# Autodesk Inventor assembly: 胴体_1
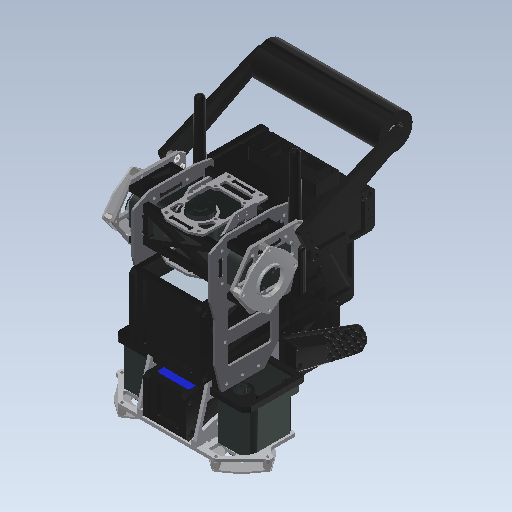
[picture p0: Inventor's stored thumbnail of the model, 512x512]
Saved by Autodesk Inventor 2020.4 (Build 244396000, 396)
## iProperties
Created: 2016-05-03
Part Number: 胴体_1
Document SubType Name: Assembly
Designer: hiroaki
Mass: 1394.39 g
Surface Area: 4542.63 cm^2
Volume: 847.153 cm^3
Density: 1.64598 g/cm^3
Author: hiroaki
## Documents named in this file (25)
- C:\Users\Masato\Documents\Inventor\CIT Brains_Inventor\OpenPlatform_ver3_0\上半身\胴体\胴体_1.iam
- C:\Users\Masato\Documents\Inventor\CIT Brains_Inventor\OpenPlatform_ver3_0\Ready_Made\B3M11xx.ipt
- C:\Users\Masato\Documents\Inventor\CIT Brains_Inventor\OpenPlatform_ver3_0\Ready_Made\B3M10xx.ipt
- C:\Users\Masato\Documents\Inventor\CIT Brains_Inventor\OpenPlatform_ver3_0\上半身\胴体\胴体_メインフレーム_1_1.ipt
- C:\Users\Masato\Documents\Inventor\CIT Brains_Inventor\OpenPlatform_ver3_0\下半身\付け根ロール\付け根ロール_サブフレーム_1_3.ipt
- C:\Users\Masato\Documents\Inventor\CIT Brains_Inventor\OpenPlatform_ver3_0\上半身\胴体\胴体_メインフレーム_1_2.ipt
- C:\Users\Masato\Documents\Inventor\CIT Brains_Inventor\OpenPlatform_ver3_0\上半身\胴体\胴体_サブフレーム_1_1.ipt
- C:\Users\Masato\Documents\Inventor\CIT Brains_Inventor\OpenPlatform_ver3_0\上半身\胴体\胴体_サブフレーム_1_2.ipt
- C:\Users\Masato\Documents\Inventor\CIT Brains_Inventor\OpenPlatform_ver3_0\上半身\胴体\胴体_サブフレーム_1_3.ipt
- C:\Users\Masato\Documents\Inventor\CIT Brains_Inventor\OpenPlatform_ver3_0\上半身\胴体\胴体_サブフレーム_1_4.ipt
- C:\Users\Masato\Documents\Inventor\CIT Brains_Inventor\OpenPlatform_ver3_0\上半身\胴体\胴体_サブフレーム_1_1_MIR.ipt
- C:\Users\Masato\Documents\Inventor\CIT Brains_Inventor\OpenPlatform_ver3_0\上半身\胴体\胴体_メインフレーム_1_12.ipt
- C:\Users\Masato\Documents\Inventor\CIT Brains_Inventor\OpenPlatform_ver3_0\上半身\胴体\胴体_メインフレーム_1_13.ipt
- C:\Users\Masato\Documents\Inventor\CIT Brains_Inventor\OpenPlatform_ver3_0\Ready_Made\MSU-306-03.ipt
- C:\Users\Masato\Documents\Inventor\CIT Brains_Inventor\OpenPlatform_ver3_0\上半身\胴体\胴体_サブフレーム_1_12.ipt
- C:\Users\Masato\Documents\Inventor\CIT Brains_Inventor\OpenPlatform_ver3_0\上半身\胴体\胴体_サブフレーム_1_4_MIR.ipt
- C:\Users\Masato\Documents\Inventor\CIT Brains_Inventor\OpenPlatform_ver3_0\上半身\胴体\RearBumper_Lower.ipt
- C:\Users\Masato\Documents\Inventor\CIT Brains_Inventor\OpenPlatform_ver3_0\上半身\胴体\RearBumper_Lower_MIR.ipt
- C:\Users\Masato\Documents\Inventor\CIT Brains_Inventor\OpenPlatform_ver3_0\Ready_Made\SGB-100.ipt
- C:\Users\Masato\Documents\Inventor\CIT Brains_Inventor\OpenPlatform_ver3_0\上半身\Cockpit\Cockpit.iam
- C:\Users\Masato\Documents\Inventor\CIT Brains_Inventor\OpenPlatform_ver3_0\Ready_Made\ASU-370H.ipt
- C:\Users\Masato\Documents\Inventor\CIT Brains_Inventor\OpenPlatform_ver3_0\Ready_Made\S3-07-3W.ipt
- C:\Users\Masato\Documents\Inventor\CIT Brains_Inventor\OpenPlatform_ver3_0\Ready_Made\SLSBF7-130-M3-N3.ipt
- C:\Users\Masato\Documents\Inventor\CIT Brains_Inventor\OpenPlatform_ver3_0\上半身\胴体\胴体_サブフレーム_改.ipt
- C:\Users\Masato\Documents\Inventor\CIT Brains_Inventor\OpenPlatform_ver3_0\上半身\胴体\胴体_サブフレーム_仮１.ipt
## Components (69 placed, 23 different names)
1. 胴体_メインフレーム_1_1:1 — 挿入:281, 挿入:282, 挿入:283, 挿入:284, 挿入:285, 挿入:286, 挿入:287, 挿入:288, 挿入:289, 挿入:290, 挿入:291, 挿入:292, 挿入:293, 挿入:294, 挿入:295, 挿入:296, 挿入:297, 挿入:298, 挿入:299, 挿入:300
2. 胴体_メインフレーム_1_2:1 — 挿入:23, 挿入:24, 挿入:25, 挿入:28, メイト:19, メイト:35
3. 胴体_サブフレーム_1_12:1 — 挿入:313, 挿入:314, 角度:55, 角度:56, 挿入:370, 角度:60
4. 胴体_サブフレーム_1_12:2 — 挿入:311, 挿入:312, 角度:57, 挿入:315, メイト:41, メイト:42, 角度:58, 角度:59
5. 胴体_メインフレーム_1_12:1 — 挿入:150, 挿入:151, 挿入:371, 挿入:372
6. 胴体_メインフレーム_1_12:2 — 挿入:162, 挿入:163, 挿入:373, 挿入:374
7. 胴体_メインフレーム_1_12:3 — 挿入:347, 挿入:348, 挿入:357, 挿入:358, 挿入:392
8. 胴体_メインフレーム_1_12:4 — 挿入:346, 挿入:349, 挿入:355, 挿入:356
9. 胴体_メインフレーム_1_13:1 — 挿入:378, 挿入:379, 挿入:380, 挿入:381
10. 胴体_メインフレーム_1_13:2 — 挿入:382, 挿入:383, 挿入:384, 挿入:385
11. 胴体_サブフレーム_1_1:1 — 挿入:275, 挿入:276, 挿入:299, 挿入:300, 角度:45, 挿入:305, 角度:51, 挿入:306, メイト:34, フラッシュ:33
12. 胴体_サブフレーム_1_1_MIR:1 — 挿入:297, 挿入:298, 挿入:301, 挿入:302, 角度:44, 挿入:303, 角度:46, 挿入:304
13. 胴体_サブフレーム_1_2:1 — フラッシュ:1, メイト:19, フラッシュ:23, フラッシュ:25, フラッシュ:28, メイト:32, メイト:35, フラッシュ:33, メイト:36, メイト:37, メイト:38, メイト:39, フラッシュ:34
14. 胴体_サブフレーム_1_2:2 — フラッシュ:1, フラッシュ:23, フラッシュ:26, フラッシュ:27, メイト:33
15. 胴体_サブフレーム_1_2:3 — フラッシュ:25, フラッシュ:28, メイト:32, メイト:34
16. 胴体_サブフレーム_1_2:4 — フラッシュ:26, フラッシュ:27, メイト:33
17. 胴体_サブフレーム_1_3:1 — 挿入:150, 挿入:151, 挿入:162, 挿入:163, 挿入:373, 挿入:374, 挿入:375, 挿入:376, 挿入:377, 挿入:378, 挿入:379, 挿入:384, 挿入:385, 挿入:394, 角度:61
18. 胴体_サブフレーム_1_3:2 — 挿入:346, 挿入:347, 挿入:348, 挿入:349, メイト:49, メイト:50, メイト:51, 挿入:380, 挿入:381, 挿入:382, 挿入:383, 挿入:392
19. 胴体_サブフレーム_1_4:1 — 挿入:57, 挿入:206, 挿入:207, 挿入:208, 挿入:209, 挿入:248, 挿入:249, 角度:53, 挿入:309, 角度:52, 挿入:310, 挿入:359, 挿入:360, 挿入:361, 挿入:371, 挿入:372
20. 胴体_サブフレーム_1_4_MIR:1 — 挿入:344, 挿入:345, 角度:50, 角度:54, 挿入:353, 挿入:354, 挿入:355, 挿入:356, 挿入:357, 挿入:358, 挿入:362, 挿入:363, 挿入:364, 挿入:365, 挿入:366, 挿入:367, 挿入:368, 挿入:369
21. 付け根ロール_サブフレーム_1_3:1 — 挿入:218, 挿入:219, 挿入:220, 挿入:221
22. 付け根ロール_サブフレーム_1_3:2 — 挿入:222, 挿入:223, 挿入:224, 挿入:225
23. 付け根ロール_サブフレーム_1_3:3 — 挿入:210, 挿入:211, 挿入:212, 挿入:213
24. 付け根ロール_サブフレーム_1_3:4 — 挿入:214, 挿入:215, 挿入:216, 挿入:217
25. 胴体_サブフレーム_改:1 — フラッシュ:35, メイト:43, メイト:44, メイト:47, メイト:48, 挿入:386, 挿入:387, 挿入:393
26. 胴体_サブフレーム_改:2 — メイト:45, フラッシュ:36, メイト:46, 挿入:388, 挿入:389, 挿入:390, 挿入:391
27. 胴体_サブフレーム_仮１:1 — メイト:47, メイト:48, フラッシュ:37
28. 胴体_サブフレーム_仮１:2 — フラッシュ:35, メイト:43, メイト:44, メイト:45, フラッシュ:36, メイト:46, フラッシュ:37, 挿入:340, 挿入:341, 挿入:342, 挿入:343
29. B3M11xx:5 — 挿入:340, 挿入:341, 挿入:342, 挿入:343
30. B3M11xx:4 — 挿入:57, 挿入:359, 挿入:360, 挿入:361, 挿入:388, 挿入:389, 挿入:390, 挿入:391
31. B3M11xx:3 — 挿入:362, 挿入:363, 挿入:364, 挿入:365, 挿入:386, 挿入:387, 挿入:393
32. B3M11xx:2 — 挿入:23, 挿入:25, 角度:23, 角度:43, 挿入:285, 挿入:286, 挿入:287, 挿入:288
33. B3M11xx:1 — 挿入:24, 挿入:28, 挿入:281, 挿入:282, 挿入:283, 挿入:284
34. MSU-306-03:1 — 挿入:218, 角度:27, 角度:29, 挿入:291
35. MSU-306-03:2 — 挿入:222, 角度:25, 角度:28, 角度:43, 挿入:296
36. MSU-306-03:3 — 挿入:220, 角度:29, 挿入:292
37. MSU-306-03:4 — 挿入:219, 角度:30, 挿入:289
38. MSU-306-03:5 — 挿入:217, 角度:34, 挿入:368
39. MSU-306-03:6 — 挿入:216, 角度:42, 挿入:369
40. MSU-306-03:7 — 挿入:225, 角度:26, 挿入:294
41. MSU-306-03:8 — 挿入:221, 角度:28, 角度:30, 挿入:290
42. MSU-306-03:9 — 挿入:206, 挿入:212, 角度:40
43. MSU-306-03:10 — 挿入:215, 角度:41, 挿入:367
44. MSU-306-03:11 — 挿入:214, 角度:33, 角度:34, 挿入:366
45. MSU-306-03:12 — 挿入:224, 角度:25, 挿入:295
46. MSU-306-03:13 — 挿入:207, 挿入:213, 角度:32
47. MSU-306-03:14 — 挿入:208, 挿入:211, 角度:32, 角度:33
48. MSU-306-03:15 — 挿入:209, 挿入:210, 角度:40, 角度:41, 角度:42
49. MSU-306-03:16 — 挿入:223, 角度:23, 角度:26, 角度:27, 挿入:293
50. MSU-306-03:17 — 挿入:313, 挿入:344, 角度:55
51. MSU-306-03:18 — 挿入:249, 挿入:312, 角度:59
52. MSU-306-03:19 — 挿入:314, 挿入:345, 角度:56
53. MSU-306-03:20 — 挿入:248, 挿入:311, 角度:58
54. RearBumper_Lower:1 — 挿入:275, 挿入:276
55. RearBumper_Lower_MIR:1 — 挿入:301, 挿入:302
56. SGB-100:1 — メイト:41, メイト:42
57. Cockpit:1 [sub-assembly] — 挿入:394, 角度:61
58. ASU-370H:1 — フラッシュ:29, フラッシュ:30, フラッシュ:31, フラッシュ:32, メイト:39, 挿入:376, メイト:51
59. ASU-370H:2 — フラッシュ:29, フラッシュ:31, メイト:36, メイト:37, フラッシュ:34, 挿入:375, メイト:49
60. ASU-370H:3 — フラッシュ:30, フラッシュ:32, メイト:38, 挿入:377, メイト:50
61. S3-07-3W:1 — 角度:44, 挿入:303
62. S3-07-3W:2 — 角度:45, 挿入:305
63. S3-07-3W:3 — 角度:46, 挿入:304
64. S3-07-3W:4 — 角度:50, 挿入:353
65. S3-07-3W:5 — 角度:51, 挿入:306
66. S3-07-3W:6 — 角度:52, 挿入:310
67. S3-07-3W:7 — 角度:53, 挿入:309
68. S3-07-3W:8 — 角度:54, 挿入:354
69. SLSBF7-130-M3-N3:1 — 角度:57, 挿入:315, 挿入:370, 角度:60
## Relationships (182: Insert 118, Angle 29, Mate 20, Flush 15)
- 挿入:23 [Insert]: 胴体_メインフレーム_1_2:1 ↔ B3M11xx:2
- 挿入:24 [Insert]: 胴体_メインフレーム_1_2:1 ↔ B3M11xx:1
- 挿入:25 [Insert]: 胴体_メインフレーム_1_2:1 ↔ B3M11xx:2
- 挿入:28 [Insert]: 胴体_メインフレーム_1_2:1 ↔ B3M11xx:1
- 挿入:57 [Insert]: 胴体_サブフレーム_1_4:1 ↔ B3M11xx:4
- 挿入:150 [Insert]: 胴体_メインフレーム_1_12:1 ↔ 胴体_サブフレーム_1_3:1
- 挿入:151 [Insert]: 胴体_メインフレーム_1_12:1 ↔ 胴体_サブフレーム_1_3:1
- 挿入:162 [Insert]: 胴体_メインフレーム_1_12:2 ↔ 胴体_サブフレーム_1_3:1
- 挿入:163 [Insert]: 胴体_メインフレーム_1_12:2 ↔ 胴体_サブフレーム_1_3:1
- 挿入:206 [Insert]: 胴体_サブフレーム_1_4:1 ↔ MSU-306-03:9
- 挿入:207 [Insert]: 胴体_サブフレーム_1_4:1 ↔ MSU-306-03:13
- 挿入:208 [Insert]: 胴体_サブフレーム_1_4:1 ↔ MSU-306-03:14
- 挿入:209 [Insert]: 胴体_サブフレーム_1_4:1 ↔ MSU-306-03:15
- 挿入:210 [Insert]: 付け根ロール_サブフレーム_1_3:3 ↔ MSU-306-03:15
- 挿入:211 [Insert]: 付け根ロール_サブフレーム_1_3:3 ↔ MSU-306-03:14
- 挿入:212 [Insert]: 付け根ロール_サブフレーム_1_3:3 ↔ MSU-306-03:9
- 挿入:213 [Insert]: 付け根ロール_サブフレーム_1_3:3 ↔ MSU-306-03:13
- 挿入:214 [Insert]: 付け根ロール_サブフレーム_1_3:4 ↔ MSU-306-03:11
- 挿入:215 [Insert]: 付け根ロール_サブフレーム_1_3:4 ↔ MSU-306-03:10
- 挿入:216 [Insert]: 付け根ロール_サブフレーム_1_3:4 ↔ MSU-306-03:6
- 挿入:217 [Insert]: 付け根ロール_サブフレーム_1_3:4 ↔ MSU-306-03:5
- 挿入:218 [Insert]: 付け根ロール_サブフレーム_1_3:1 ↔ MSU-306-03:1
- 挿入:219 [Insert]: 付け根ロール_サブフレーム_1_3:1 ↔ MSU-306-03:4
- 挿入:220 [Insert]: 付け根ロール_サブフレーム_1_3:1 ↔ MSU-306-03:3
- 挿入:221 [Insert]: 付け根ロール_サブフレーム_1_3:1 ↔ MSU-306-03:8
- 挿入:222 [Insert]: 付け根ロール_サブフレーム_1_3:2 ↔ MSU-306-03:2
- 挿入:223 [Insert]: 付け根ロール_サブフレーム_1_3:2 ↔ MSU-306-03:16
- 挿入:224 [Insert]: 付け根ロール_サブフレーム_1_3:2 ↔ MSU-306-03:12
- 挿入:225 [Insert]: 付け根ロール_サブフレーム_1_3:2 ↔ MSU-306-03:7
- 角度:23 [Angle] (0 deg): B3M11xx:2 ↔ MSU-306-03:16
- 角度:25 [Angle] (0 deg): MSU-306-03:2 ↔ MSU-306-03:12
- 角度:26 [Angle] (0 deg): MSU-306-03:7 ↔ MSU-306-03:16
- 角度:27 [Angle] (0 deg): MSU-306-03:1 ↔ MSU-306-03:16
- 角度:28 [Angle] (0 deg): MSU-306-03:2 ↔ MSU-306-03:8
- 角度:29 [Angle] (0 deg): MSU-306-03:1 ↔ MSU-306-03:3
- 角度:30 [Angle] (0 deg): MSU-306-03:4 ↔ MSU-306-03:8
- 角度:32 [Angle] (0 deg): MSU-306-03:13 ↔ MSU-306-03:14
- 角度:33 [Angle] (0 deg): MSU-306-03:11 ↔ MSU-306-03:14
- 角度:34 [Angle] (0 deg): MSU-306-03:5 ↔ MSU-306-03:11
- フラッシュ:1 [Flush]: 胴体_サブフレーム_1_2:1 ↔ 胴体_サブフレーム_1_2:2
- 挿入:248 [Insert]: 胴体_サブフレーム_1_4:1 ↔ MSU-306-03:20
- 挿入:249 [Insert]: 胴体_サブフレーム_1_4:1 ↔ MSU-306-03:18
- 角度:40 [Angle] (0 deg): MSU-306-03:9 ↔ MSU-306-03:15
- 角度:41 [Angle] (0 deg): MSU-306-03:10 ↔ MSU-306-03:15
- 角度:42 [Angle] (0 deg): MSU-306-03:6 ↔ MSU-306-03:15
- 角度:43 [Angle] (0 deg): B3M11xx:2 ↔ MSU-306-03:2
- 挿入:275 [Insert]: 胴体_サブフレーム_1_1:1 ↔ RearBumper_Lower:1
- 挿入:276 [Insert]: 胴体_サブフレーム_1_1:1 ↔ RearBumper_Lower:1
- 挿入:281 [Insert]: 胴体_メインフレーム_1_1:1 ↔ B3M11xx:1
- 挿入:282 [Insert]: 胴体_メインフレーム_1_1:1 ↔ B3M11xx:1
- 挿入:283 [Insert]: 胴体_メインフレーム_1_1:1 ↔ B3M11xx:1
- 挿入:284 [Insert]: 胴体_メインフレーム_1_1:1 ↔ B3M11xx:1
- 挿入:285 [Insert]: 胴体_メインフレーム_1_1:1 ↔ B3M11xx:2
- 挿入:286 [Insert]: 胴体_メインフレーム_1_1:1 ↔ B3M11xx:2
- 挿入:287 [Insert]: 胴体_メインフレーム_1_1:1 ↔ B3M11xx:2
- 挿入:288 [Insert]: 胴体_メインフレーム_1_1:1 ↔ B3M11xx:2
- 挿入:289 [Insert]: 胴体_メインフレーム_1_1:1 ↔ MSU-306-03:4
- 挿入:290 [Insert]: 胴体_メインフレーム_1_1:1 ↔ MSU-306-03:8
- 挿入:291 [Insert]: 胴体_メインフレーム_1_1:1 ↔ MSU-306-03:1
- 挿入:292 [Insert]: 胴体_メインフレーム_1_1:1 ↔ MSU-306-03:3
- 挿入:293 [Insert]: 胴体_メインフレーム_1_1:1 ↔ MSU-306-03:16
- 挿入:294 [Insert]: 胴体_メインフレーム_1_1:1 ↔ MSU-306-03:7
- 挿入:295 [Insert]: 胴体_メインフレーム_1_1:1 ↔ MSU-306-03:12
- 挿入:296 [Insert]: 胴体_メインフレーム_1_1:1 ↔ MSU-306-03:2
- 挿入:297 [Insert]: 胴体_メインフレーム_1_1:1 ↔ 胴体_サブフレーム_1_1_MIR:1
- 挿入:298 [Insert]: 胴体_メインフレーム_1_1:1 ↔ 胴体_サブフレーム_1_1_MIR:1
- 挿入:299 [Insert]: 胴体_メインフレーム_1_1:1 ↔ 胴体_サブフレーム_1_1:1
- 挿入:300 [Insert]: 胴体_メインフレーム_1_1:1 ↔ 胴体_サブフレーム_1_1:1
- 挿入:301 [Insert]: 胴体_サブフレーム_1_1_MIR:1 ↔ RearBumper_Lower_MIR:1
- 挿入:302 [Insert]: 胴体_サブフレーム_1_1_MIR:1 ↔ RearBumper_Lower_MIR:1
- メイト:19 [Mate]: 胴体_メインフレーム_1_2:1 ↔ 胴体_サブフレーム_1_2:1
- フラッシュ:23 [Flush]: 胴体_サブフレーム_1_2:1 ↔ 胴体_サブフレーム_1_2:2
- 角度:44 [Angle] (0 deg): 胴体_サブフレーム_1_1_MIR:1 ↔ S3-07-3W:1
- 挿入:303 [Insert]: 胴体_サブフレーム_1_1_MIR:1 ↔ S3-07-3W:1
- 角度:46 [Angle] (0 deg): 胴体_サブフレーム_1_1_MIR:1 ↔ S3-07-3W:3
- 挿入:304 [Insert]: 胴体_サブフレーム_1_1_MIR:1 ↔ S3-07-3W:3
- 角度:45 [Angle] (0 deg): 胴体_サブフレーム_1_1:1 ↔ S3-07-3W:2
- 挿入:305 [Insert]: 胴体_サブフレーム_1_1:1 ↔ S3-07-3W:2
- 角度:51 [Angle] (0 deg): 胴体_サブフレーム_1_1:1 ↔ S3-07-3W:5
- 挿入:306 [Insert]: 胴体_サブフレーム_1_1:1 ↔ S3-07-3W:5
- 角度:53 [Angle] (0 deg): 胴体_サブフレーム_1_4:1 ↔ S3-07-3W:7
- 挿入:309 [Insert]: 胴体_サブフレーム_1_4:1 ↔ S3-07-3W:7
- 角度:52 [Angle] (0 deg): 胴体_サブフレーム_1_4:1 ↔ S3-07-3W:6
- 挿入:310 [Insert]: 胴体_サブフレーム_1_4:1 ↔ S3-07-3W:6
- フラッシュ:25 [Flush]: 胴体_サブフレーム_1_2:1 ↔ 胴体_サブフレーム_1_2:3
- フラッシュ:26 [Flush]: 胴体_サブフレーム_1_2:2 ↔ 胴体_サブフレーム_1_2:4
- フラッシュ:27 [Flush]: 胴体_サブフレーム_1_2:2 ↔ 胴体_サブフレーム_1_2:4
- フラッシュ:28 [Flush]: 胴体_サブフレーム_1_2:1 ↔ 胴体_サブフレーム_1_2:3
- メイト:32 [Mate]: 胴体_サブフレーム_1_2:1 ↔ 胴体_サブフレーム_1_2:3
- メイト:33 [Mate]: 胴体_サブフレーム_1_2:2 ↔ 胴体_サブフレーム_1_2:4
- メイト:34 [Mate]: 胴体_サブフレーム_1_1:1 ↔ 胴体_サブフレーム_1_2:3
- フラッシュ:29 [Flush]: ASU-370H:1 ↔ ASU-370H:2
- フラッシュ:30 [Flush]: ASU-370H:1 ↔ ASU-370H:3
- フラッシュ:31 [Flush]: ASU-370H:1 ↔ ASU-370H:2
- フラッシュ:32 [Flush]: ASU-370H:1 ↔ ASU-370H:3
- メイト:35 [Mate]: 胴体_メインフレーム_1_2:1 ↔ 胴体_サブフレーム_1_2:1
- フラッシュ:33 [Flush]: 胴体_サブフレーム_1_1:1 ↔ 胴体_サブフレーム_1_2:1
- メイト:36 [Mate] (0.01 mm): 胴体_サブフレーム_1_2:1 ↔ ASU-370H:2
- メイト:37 [Mate] (0.01 mm): 胴体_サブフレーム_1_2:1 ↔ ASU-370H:2
- メイト:38 [Mate] (0.01 mm): 胴体_サブフレーム_1_2:1 ↔ ASU-370H:3
- メイト:39 [Mate] (0.01 mm): 胴体_サブフレーム_1_2:1 ↔ ASU-370H:1
- フラッシュ:34 [Flush]: 胴体_サブフレーム_1_2:1 ↔ ASU-370H:2
- 挿入:311 [Insert]: 胴体_サブフレーム_1_12:2 ↔ MSU-306-03:20
- 挿入:312 [Insert]: 胴体_サブフレーム_1_12:2 ↔ MSU-306-03:18
- 挿入:313 [Insert]: 胴体_サブフレーム_1_12:1 ↔ MSU-306-03:17
- 挿入:314 [Insert]: 胴体_サブフレーム_1_12:1 ↔ MSU-306-03:19
- 角度:57 [Angle] (0 deg): 胴体_サブフレーム_1_12:2 ↔ SLSBF7-130-M3-N3:1
- 挿入:315 [Insert]: 胴体_サブフレーム_1_12:2 ↔ SLSBF7-130-M3-N3:1
- メイト:41 [Mate]: 胴体_サブフレーム_1_12:2 ↔ SGB-100:1
- メイト:42 [Mate]: 胴体_サブフレーム_1_12:2 ↔ SGB-100:1
- フラッシュ:35 [Flush]: 胴体_サブフレーム_改:1 ↔ 胴体_サブフレーム_仮１:2
- メイト:43 [Mate] (0.01 mm): 胴体_サブフレーム_改:1 ↔ 胴体_サブフレーム_仮１:2
- メイト:44 [Mate] (0.01 mm): 胴体_サブフレーム_改:1 ↔ 胴体_サブフレーム_仮１:2
- メイト:45 [Mate] (0.01 mm): 胴体_サブフレーム_改:2 ↔ 胴体_サブフレーム_仮１:2
- フラッシュ:36 [Flush]: 胴体_サブフレーム_改:2 ↔ 胴体_サブフレーム_仮１:2
- メイト:46 [Mate] (0.01 mm): 胴体_サブフレーム_改:2 ↔ 胴体_サブフレーム_仮１:2
- メイト:47 [Mate] (0.01 mm): 胴体_サブフレーム_改:1 ↔ 胴体_サブフレーム_仮１:1
- メイト:48 [Mate] (0.01 mm): 胴体_サブフレーム_改:1 ↔ 胴体_サブフレーム_仮１:1
- フラッシュ:37 [Flush]: 胴体_サブフレーム_仮１:1 ↔ 胴体_サブフレーム_仮１:2
- 挿入:340 [Insert]: 胴体_サブフレーム_仮１:2 ↔ B3M11xx:5
- 挿入:341 [Insert]: 胴体_サブフレーム_仮１:2 ↔ B3M11xx:5
- 挿入:342 [Insert]: 胴体_サブフレーム_仮１:2 ↔ B3M11xx:5
- 挿入:343 [Insert]: 胴体_サブフレーム_仮１:2 ↔ B3M11xx:5
- 挿入:344 [Insert]: 胴体_サブフレーム_1_4_MIR:1 ↔ MSU-306-03:17
- 挿入:345 [Insert]: 胴体_サブフレーム_1_4_MIR:1 ↔ MSU-306-03:19
- 挿入:346 [Insert]: 胴体_メインフレーム_1_12:4 ↔ 胴体_サブフレーム_1_3:2
- 挿入:347 [Insert]: 胴体_メインフレーム_1_12:3 ↔ 胴体_サブフレーム_1_3:2
- 挿入:348 [Insert]: 胴体_メインフレーム_1_12:3 ↔ 胴体_サブフレーム_1_3:2
- 挿入:349 [Insert]: 胴体_メインフレーム_1_12:4 ↔ 胴体_サブフレーム_1_3:2
- 角度:50 [Angle] (0 deg): 胴体_サブフレーム_1_4_MIR:1 ↔ S3-07-3W:4
- 角度:54 [Angle] (0 deg): 胴体_サブフレーム_1_4_MIR:1 ↔ S3-07-3W:8
- 挿入:353 [Insert]: 胴体_サブフレーム_1_4_MIR:1 ↔ S3-07-3W:4
- 挿入:354 [Insert]: 胴体_サブフレーム_1_4_MIR:1 ↔ S3-07-3W:8
- 挿入:355 [Insert]: 胴体_メインフレーム_1_12:4 ↔ 胴体_サブフレーム_1_4_MIR:1
- 挿入:356 [Insert]: 胴体_メインフレーム_1_12:4 ↔ 胴体_サブフレーム_1_4_MIR:1
- 挿入:357 [Insert]: 胴体_メインフレーム_1_12:3 ↔ 胴体_サブフレーム_1_4_MIR:1
- 挿入:358 [Insert]: 胴体_メインフレーム_1_12:3 ↔ 胴体_サブフレーム_1_4_MIR:1
- 挿入:359 [Insert]: 胴体_サブフレーム_1_4:1 ↔ B3M11xx:4
- 挿入:360 [Insert]: 胴体_サブフレーム_1_4:1 ↔ B3M11xx:4
- 挿入:361 [Insert]: 胴体_サブフレーム_1_4:1 ↔ B3M11xx:4
- 挿入:362 [Insert]: 胴体_サブフレーム_1_4_MIR:1 ↔ B3M11xx:3
- 挿入:363 [Insert]: 胴体_サブフレーム_1_4_MIR:1 ↔ B3M11xx:3
- 挿入:364 [Insert]: 胴体_サブフレーム_1_4_MIR:1 ↔ B3M11xx:3
- 挿入:365 [Insert]: 胴体_サブフレーム_1_4_MIR:1 ↔ B3M11xx:3
- 挿入:366 [Insert]: 胴体_サブフレーム_1_4_MIR:1 ↔ MSU-306-03:11
- 挿入:367 [Insert]: 胴体_サブフレーム_1_4_MIR:1 ↔ MSU-306-03:10
- 挿入:368 [Insert]: 胴体_サブフレーム_1_4_MIR:1 ↔ MSU-306-03:5
- 挿入:369 [Insert]: 胴体_サブフレーム_1_4_MIR:1 ↔ MSU-306-03:6
- 角度:55 [Angle] (0 deg): 胴体_サブフレーム_1_12:1 ↔ MSU-306-03:17
- 角度:56 [Angle] (0 deg): 胴体_サブフレーム_1_12:1 ↔ MSU-306-03:19
- 角度:58 [Angle] (0 deg): 胴体_サブフレーム_1_12:2 ↔ MSU-306-03:20
- 角度:59 [Angle] (0 deg): 胴体_サブフレーム_1_12:2 ↔ MSU-306-03:18
- 挿入:370 [Insert]: 胴体_サブフレーム_1_12:1 ↔ SLSBF7-130-M3-N3:1
- 挿入:371 [Insert]: 胴体_メインフレーム_1_12:1 ↔ 胴体_サブフレーム_1_4:1
- 挿入:372 [Insert]: 胴体_メインフレーム_1_12:1 ↔ 胴体_サブフレーム_1_4:1
- 挿入:373 [Insert]: 胴体_メインフレーム_1_12:2 ↔ 胴体_サブフレーム_1_3:1
- 挿入:374 [Insert]: 胴体_メインフレーム_1_12:2 ↔ 胴体_サブフレーム_1_3:1
- 角度:60 [Angle] (0 deg): 胴体_サブフレーム_1_12:1 ↔ SLSBF7-130-M3-N3:1
- 挿入:375 [Insert]: 胴体_サブフレーム_1_3:1 ↔ ASU-370H:2
- 挿入:376 [Insert]: 胴体_サブフレーム_1_3:1 ↔ ASU-370H:1
- 挿入:377 [Insert]: 胴体_サブフレーム_1_3:1 ↔ ASU-370H:3
- メイト:49 [Mate]: 胴体_サブフレーム_1_3:2 ↔ ASU-370H:2
- メイト:50 [Mate]: 胴体_サブフレーム_1_3:2 ↔ ASU-370H:3
- メイト:51 [Mate]: 胴体_サブフレーム_1_3:2 ↔ ASU-370H:1
- 挿入:378 [Insert]: 胴体_メインフレーム_1_13:1 ↔ 胴体_サブフレーム_1_3:1
- 挿入:379 [Insert]: 胴体_メインフレーム_1_13:1 ↔ 胴体_サブフレーム_1_3:1
- 挿入:380 [Insert]: 胴体_メインフレーム_1_13:1 ↔ 胴体_サブフレーム_1_3:2
- 挿入:381 [Insert]: 胴体_メインフレーム_1_13:1 ↔ 胴体_サブフレーム_1_3:2
- 挿入:382 [Insert]: 胴体_メインフレーム_1_13:2 ↔ 胴体_サブフレーム_1_3:2
- 挿入:383 [Insert]: 胴体_メインフレーム_1_13:2 ↔ 胴体_サブフレーム_1_3:2
- 挿入:384 [Insert]: 胴体_メインフレーム_1_13:2 ↔ 胴体_サブフレーム_1_3:1
- 挿入:385 [Insert]: 胴体_メインフレーム_1_13:2 ↔ 胴体_サブフレーム_1_3:1
- 挿入:386 [Insert]: 胴体_サブフレーム_改:1 ↔ B3M11xx:3
- 挿入:387 [Insert]: 胴体_サブフレーム_改:1 ↔ B3M11xx:3
- 挿入:388 [Insert]: 胴体_サブフレーム_改:2 ↔ B3M11xx:4
- 挿入:389 [Insert]: 胴体_サブフレーム_改:2 ↔ B3M11xx:4
- 挿入:390 [Insert]: 胴体_サブフレーム_改:2 ↔ B3M11xx:4
- 挿入:391 [Insert]: 胴体_サブフレーム_改:2 ↔ B3M11xx:4
- 挿入:392 [Insert]: 胴体_メインフレーム_1_12:3 ↔ 胴体_サブフレーム_1_3:2
- 挿入:393 [Insert]: 胴体_サブフレーム_改:1 ↔ B3M11xx:3
- 挿入:394 [Insert] (2 mm): 胴体_サブフレーム_1_3:1 ↔ Cockpit:1
- 角度:61 [Angle] (0 deg): 胴体_サブフレーム_1_3:1 ↔ Cockpit:1
